# Autodesk Inventor assembly: Garage_Simplified
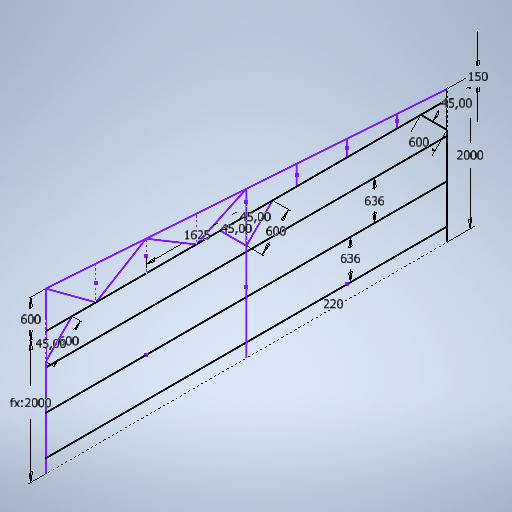
[picture p0: Inventor's stored thumbnail of the model, 512x512]
Saved by Autodesk Inventor 2025.2 (Build 292293000, 293)
## iProperties
Created: 2025-09-29
Part Number: Garage_Simplified
Document SubType Name: Assembly
Designer: MB
_SolveAssemblyDoc: Frame Generator Solve Assembly
_Version: 15.0.0
Author: MB
## iProperties of the stored document MemberDocs/x50qknvc4B05kgkevHifztjknEb
_SolveAssemblyDoc: Frame Generator Solve Assembly
_Version: 15.0.0
Created: 2025-09-29
Part Number: Garage_Simplified
Document SubType Name: Assembly
Designer: MB
Mass: 535689 g
Surface Area: 431223 cm^2
Volume: 68249.9 cm^3
Density: 7.84893 g/cm^3
Author: MB
## Documents named in this file (10)
- C:\Users\Catch22\Documents\Github\hegesztes\Garage_Simplified.iam
- C:\Users\MB\Documents\GitHub\hegesztes\Garage_40x40.ipt
- C:\Users\MB\Documents\GitHub\hegesztes\Garage_Simplified\Frame\Frame 1759173587755.iam
- C:\Users\Catch22\Documents\Github\hegesztes\Garage_40x40.ipt
- C:\Users\Catch22\Documents\Github\hegesztes\Garage_Simplified\Frame\Frame 1759173587755.iam
- C:\Users\Catch22\Documents\Github\hegesztes\Front_Truss.iam
- C:\Users\Catch22\Documents\Github\hegesztes\TopNew.iam
- C:\Users\Catch22\Documents\Github\hegesztes\RearNew.iam
- C:\Users\Catch22\Documents\Github\hegesztes\MiddleTruss.iam
- C:\Users\Catch22\Documents\Github\hegesztes\LVas.ipt
## Components (3 placed, 2 different names)
1. Garage_40x40:1
2. Frame 1759173587755:1 [sub-assembly]
3. Frame 1759173587755:3 [sub-assembly]
## Component patterns: (2 elements, first: Frame 1759173587755:1)
